# Autodesk Inventor assembly: LaundryRobot_v01
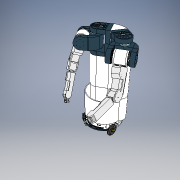
[picture p0: Inventor's stored thumbnail of the model, 180x180]
Saved by Autodesk Inventor 2017 SP1 (Build 210196100, 196)
## iProperties
Created: 2017-03-11
Part Number: LaundryRobot_v01
Document SubType Name: Assembly
Designer: zallen
Author: zallen
## Documents named in this file (3)
- C:\Users\Zach\Documents\GitHub\cr-laundry-robot\LaundryRobot_v01.iam
- C:\Users\Zach\Documents\GitHub\cr-laundry-robot\src\Base\Base.iam
- C:\Users\Zach\Documents\GitHub\cr-laundry-robot\src\Body\Body.iam
## Components (2 placed, 2 different names)
1. Base:1 [sub-assembly] — Mate:1, Mate:2, Mate:4, Mate:5, Mate:6
2. Body:1 [sub-assembly] — Mate:1, Mate:2, Mate:7, Mate:8
## Relationships (7: Mate 7)
- Mate:1: Base:1 ↔ Body:1
- Mate:2: Base:1 ↔ Body:1
- Mate:4: Base:1
- Mate:5: Base:1
- Mate:6: Base:1
- Mate:7: Body:1
- Mate:8: Body:1
